# Autodesk Inventor assembly: Pump-Motor-CW-Rotation:Motor CW
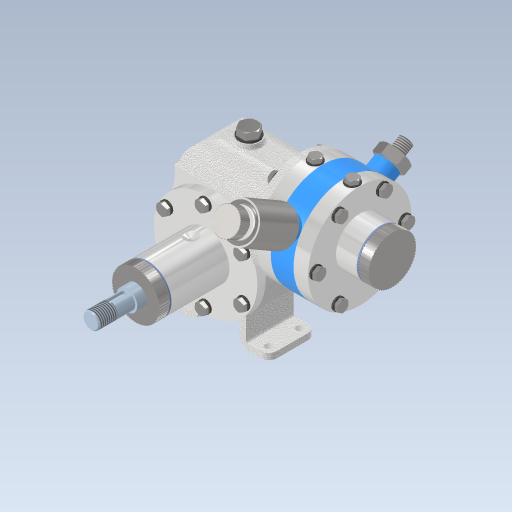
[picture p0: Inventor's stored thumbnail of the model, 512x512]
Saved by Autodesk Inventor 2024.2 (Build 282272000, 272)
## iProperties
Created: 2025-06-16
Document SubType Name: Assembly
Designer: cw
Description: Motor CW
Author: cw
## Documents named in this file (42)
- C:\zWSA2025 TP05 M1\Solution\Motor Final CW.iam
- C:\zWSA2025 TP05 M1\Solution\Motor\Housing.ipt
- C:\zWSA2025 TP05 M1\Solution\Design Accelerator\Worm Gears1.iam
- C:\zWSA2025 TP05 M1\Solution\Motor\Casing 101.ipt
- C:\zWSA2025 TP05 M1\Solution\Motor\Bush.ipt
- C:\zWSA2025 TP05 M1\Solution\Motor\Shaft.ipt
- C:\zWSA2025 TP05 M1\Solution\Motor\Cover 102.ipt
- C:\zWSA2025 TP05 M1\Solution\Motor\Gasket 103.ipt
- C:\zWSA2025 TP05 M1\Solution\Motor\Seal Ring.ipt
- C:\zWSA2025 TP05 M1\Solution\Content Center\en-US\DIN 6885-1 A\DIN 6885 - A 4 x 4 x 25.ipt
- C:\zWSA2025 TP05 M1\Solution\Motor\Washer.ipt
- C:\zWSA2025 TP05 M1\Solution\Motor\Lock Nut.ipt
- C:\zWSA2025\M1\Casing 103 config.ipt
- C:\zWSA2025 TP05 M1\Solution\Content Center\en-US\DIN 3760 A\DIN 3760 - A - 14 x 24 x 7 - NBR.ipt
- C:\zWSA2025 TP05 M1\Solution\Content Center\en-US\DIN 472(1)\DIN 472 - 24 x 1.2.ipt
- C:\zWSA2025 TP05 M1\Solution\Content Center\en-US\DIN 625 SKF(5)\DIN 625 SKF - SKF 6001-2RSH.ipt
- C:\zWSA2025 TP05 M1\Solution\Motor\Spacer.ipt
- C:\zWSA2025 TP05 M1\Solution\Drive Shaft.ipt
- C:\zWSA2025 TP05 M1\Solution\Content Center\en-US\DIN 6885-1 A\DIN 6885 - A 4 x 4 x 28.ipt
- C:\zWSA2025 TP05 M1\Solution\Motor\M Case.ipt
- C:\zWSA2025 TP05 M1\Solution\Content Center\en-US\DIN 6885-1 A\DIN 6885 - A 5 x 5 x 18.ipt
- C:\zWSA2025 TP05 M1\Solution\Motor\Rotor.ipt
- C:\zWSA2025 TP05 M1\Solution\Motor\Vane.ipt
- C:\zWSA2025 TP05 M1\Solution\Content Center\en-US\ISO 8734(2)\ISO 8734 - 5 x 30 - AISO (2).ipt
- C:\zWSA2025\M1\Casing 102 config.ipt
- C:\zWSA2025 TP05 M1\Solution\Motor\Cover 101.ipt
- C:\zWSA2025 TP05 M1\Solution\Motor\Port.ipt
- C:\zWSA2025 TP05 M1\Solution\Motor\S Barrel.ipt
- C:\zWSA2025 TP05 M1\Solution\Motor\Cap 101.ipt
- C:\zWSA2025 TP05 M1\Solution\Content Center\en-US\ISO 4035(2)\ISO 4035 - M12 - ISO.ipt
- C:\zWSA2025 TP05 M1\Solution\Motor\Cap 102.ipt
- C:\zWSA2025 TP05 M1\Solution\Motor\Cover 103.ipt
- C:\zWSA2025 TP05 M1\Solution\Content Center\en-US\ISO 4017(1)\ISO 4017 - M6 x 16 - ISO.ipt
- C:\zWSA2025 TP05 M1\Solution\Content Center\en-US\ISO 7091\ISO 7091 - ST 6 - 100 HV.ipt
- C:\zWSA2025 TP05 M1\Solution\Content Center\en-US\ISO 4017(1)\ISO 4017 - M6 x 30 - ISO.ipt
- C:\zWSA2025 TP05 M1\Solution\Content Center\en-US\ISO 4017(1)\ISO 4017 - M6 x 25 - ISO.ipt
- C:\zWSA2025 TP05 M1\Solution\Motor\Plug 101.ipt
- C:\zWSA2025 TP05 M1\Solution\Motor\Gasket 101.ipt
- C:\zWSA2025 TP05 M1\Solution\Motor\Plug 102.ipt
- C:\zWSA2025 TP05 M1\Solution\Motor\Gasket 102.ipt
- C:\zWSA2025 TP05 M1\Solution\Casing 103 config\Casing 103-cw.ipt
- C:\zWSA2025 TP05 M1\Solution\Casing 102 config\Casing 102-cw.ipt
## Components (88 placed, 39 different names)
1. Housing:1 — Mate:3, Mate:4, Mate:21, Angle:1(RotateDriveDrive), Mate:30, Mate:31, Mate:32, Mate:33, Mate:34, Flush:7(4cw), Mate:61(4ccw), Mate:114, Mate:115, Angle:103, Angle:104, Mate:134, Mate:135, Angle:108, Mate:138, Mate:139, Angle:109, Angle:110(RotateShaft)
2. Worm Gears:1 [sub-assembly] — Flush:2, Mate:26, Mate:30, Mate:31, Mate:45, Flush:5, Mate:53
3. Casing 101:1 — Mate:3, Mate:4, Mate:5, Mate:6, Mate:7, Mate:8, Mate:9, Mate:10, Mate:11, Mate:18, Mate:19, Mate:20, Mate:21, Mate:110, Mate:111, Angle:102
4. Bush:1 — Mate:5, Mate:6, Mate:7
5. Bush:2 — Mate:8, Mate:9, Mate:10, Mate:12
6. Shaft:1 — Mate:11, Mate:12, Mate:22, Mate:23, Mate:24, Flush:2, Mate:25, Mate:27, Mate:28, Angle:110(RotateShaft)
7. Cover 102:1 — Mate:13, Mate:14, Mate:15, Mate:16, Flush:1, Mate:17, Mate:18, Mate:20
8. Gasket 103:1 — Mate:13, Mate:14, Mate:15, Mate:19
9. Seal Ring:1 — Mate:16, Flush:1, Mate:17
10. DIN 6885-1 A A 4 x 4 x 25:1 — Mate:22, Mate:23, Mate:24
11. Washer:1 — Mate:25, Mate:26, Mate:27, Mate:29, Flush:3
12. Lock Nut:1 — Mate:28, Mate:29, Flush:3
13. Casing 103-cw:1 — Mate:32, Mate:33, Mate:34, Mate:38, Mate:39, Mate:41, Flush:4, Mate:40, Mate:43, Mate:44, Mate:58(4cw), Mate:60(4ccw), Mate:79, Mate:80, Mate:118, Mate:119, Mate:126, Mate:127, Angle:106
14. DIN 3760 A A - 14 x 24 x 7 - NBR:1 — Mate:35, Mate:36, Mate:37, Mate:38, Mate:39, Mate:40
15. DIN 3760 A A - 14 x 24 x 7 - NBR:2 — Mate:35, Mate:36, Mate:37, Mate:42
16. DIN 472 24 x 1.2:1 — Mate:41, Mate:42, Flush:4
17. DIN 625 SKF- with two RS1 seals SKF 6001-2RSH:1 — Mate:43, Mate:44, Mate:47, Mate:48, Flush:6
18. Spacer:1 — Mate:46, Mate:47
19. Drive Shaft:1 — Mate:45, Mate:46, Mate:48, Flush:5, Flush:6, Mate:49, Mate:50, Mate:51, Mate:52, Mate:54, Mate:55, Angle:1(RotateDriveDrive), Mate:59(4cw), Flush:8(4ccw), Mate:62, Mate:63, Mate:64, Mate:65(4cw), Flush:9(4cw), Flush:10(4cw), Mate:66(4ccw), Mate:67(4ccw), Mate:68(4ccw), Mate:78, Mate:81, Mate:82, Mate:84, Mate:85, Mate:87
20. DIN 6885-1 A A 4 x 4 x 28:1 — Mate:49, Mate:50, Mate:51
21. Washer:2 — Mate:52, Mate:53, Mate:54, Mate:56, Mate:57
22. Lock Nut:2 — Mate:55, Mate:56, Mate:57
23. M Case:1 — Mate:58(4cw), Mate:59(4cw), Flush:7(4cw), Mate:60(4ccw), Flush:8(4ccw), Mate:61(4ccw), Tangent:1(4cw), Tangent:2 (4ccw), Tangent:3(4cw), Tangent:4(4ccw), Tangent:5(4cw), Tangent:6(4ccw), Tangent:7(4cw), Tangent:8(4ccw), Mate:74, Flush:83, Mate:75, Flush:84, Mate:94, Mate:95, Angle:97, Mate:96, Mate:97, Angle:98, Mate:99
24. DIN 6885-1 A A 5 x 5 x 18:1 — Mate:62, Mate:63, Mate:64
25. Rotor:1 — Mate:65(4cw), Flush:9(4cw), Flush:10(4cw), Mate:66(4ccw), Mate:67(4ccw), Mate:68(4ccw), Flush:70(4cw), Mate:70(4cw), Flush:72(4ccw), Mate:71(4ccw), Flush:73(4cw), Mate:72(4cw), Flush:74(4ccw), Flush:75(4ccw), Flush:76(4cw), Flush:77(4cw), Flush:78(4ccw), Flush:79(4ccw), Flush:80(4cw), Flush:81(4cw), Flush:82(4ccw), Mate:73(4ccw)
26. Vane:1 — Flush:70(4cw), Mate:70(4cw), Tangent:1(4cw), Flush:72(4ccw), Mate:71(4ccw), Tangent:2 (4ccw)
27. Vane:2 — Flush:73(4cw), Mate:72(4cw), Tangent:3(4cw), Flush:74(4ccw), Flush:75(4ccw), Tangent:4(4ccw)
28. Vane:3 — Flush:76(4cw), Flush:77(4cw), Tangent:5(4cw), Flush:78(4ccw), Flush:79(4ccw), Tangent:6(4ccw)
29. Vane:4 — Flush:80(4cw), Flush:81(4cw), Tangent:7(4cw), Flush:82(4ccw), Mate:73(4ccw), Tangent:8(4ccw)
30. ISO 8734 5 x 30 - A:1 — Mate:74, Flush:83
31. ISO 8734 5 x 30 - A:2 — Mate:75, Flush:84
32. Casing 102-cw:1 — Mate:76, Mate:77, Mate:78, Mate:79, Mate:80, Mate:91, Mate:92, Mate:93, Mate:122, Mate:123, Angle:105, Mate:130, Mate:131, Angle:107
33. DIN 625 SKF- with two RS1 seals SKF 6001-2RSH:2 — Mate:76, Mate:77, Mate:81, Mate:83
34. Washer:3 — Mate:82, Mate:83, Mate:84, Mate:86
35. Lock Nut:3 — Mate:85, Mate:86, Mate:87
36. Gasket 103:2 — Mate:88, Mate:89, Mate:90, Mate:92
37. Cover 101:1 — Mate:88, Mate:89, Mate:90, Mate:91, Mate:93
38. Port:1 — Mate:94, Mate:95, Angle:97
39. S Barrel:1 — Mate:96, Mate:97, Angle:98, Mate:98, Mate:100, Angle:99, Mate:102, Mate:103, Angle:100, Mate:104, Mate:106, Angle:101
40. Cap 101:1 — Mate:98, Mate:99, Mate:101
41. ISO 4035 M12:1 — Mate:100, Mate:101, Angle:99
42. ISO 4035 M12:2 — Mate:102, Mate:103, Angle:100, Mate:105
43. Cap 102:1 — Mate:104, Mate:105, Mate:107
44. Cover 103:1 — Mate:106, Mate:107, Angle:101
45. Plug 101:1 — Mate:124, Mate:125, Mate:126, Angle:106
46. Plug 101:2 — Mate:128, Mate:129, Mate:130, Angle:107
47. Gasket 101:1 — Mate:124, Mate:125, Mate:127
48. Gasket 101:2 — Mate:128, Mate:129, Mate:131
49. Plug 102:1 — Mate:132, Mate:133, Mate:134, Angle:108
50. Plug 102:2 — Mate:136, Mate:137, Mate:138, Angle:109
51. Gasket 102:1 — Mate:132, Mate:133, Mate:135
52. Gasket 102:2 — Mate:136, Mate:137, Mate:139
53. ISO 4017 M6 x 16:1 — Mate:108, Mate:109, Mate:110, Angle:102
54. ISO 7091 ST 6 - 100 HV:1 — Mate:108, Mate:109, Mate:111
55. ISO 4017 M6 x 16:2
56. ISO 7091 ST 6 - 100 HV:2
57. ISO 4017 M6 x 16:3
58. ISO 7091 ST 6 - 100 HV:3
59. ISO 4017 M6 x 16:4
60. ISO 7091 ST 6 - 100 HV:4
61. ISO 4017 M6 x 16:5
62. ISO 7091 ST 6 - 100 HV:5
63. ISO 4017 M6 x 16:6
64. ISO 7091 ST 6 - 100 HV:6
65. ISO 4017 M6 x 30:1 — Mate:112, Mate:113, Mate:114, Angle:103
66. ISO 7091 ST 6 - 100 HV:7 — Mate:112, Mate:113, Mate:115
67. ISO 4017 M6 x 30:2
68. ISO 7091 ST 6 - 100 HV:8
69. ISO 4017 M6 x 30:3
70. ISO 7091 ST 6 - 100 HV:9
71. ISO 4017 M6 x 30:4
72. ISO 7091 ST 6 - 100 HV:10
73. ISO 4017 M6 x 25:1 — Mate:116, Mate:117, Mate:118, Angle:104
74. ISO 7091 ST 6 - 100 HV:11 — Mate:116, Mate:117, Mate:119
75. ISO 4017 M6 x 25:2
76. ISO 7091 ST 6 - 100 HV:12
77. ISO 4017 M6 x 25:3 — Mate:120, Mate:121, Mate:122, Angle:105
78. ISO 7091 ST 6 - 100 HV:13 — Mate:120, Mate:121, Mate:123
79. ISO 4017 M6 x 25:4
80. ISO 7091 ST 6 - 100 HV:14
81. ISO 4017 M6 x 25:5
82. ISO 7091 ST 6 - 100 HV:15
83. ISO 4017 M6 x 25:6
84. ISO 7091 ST 6 - 100 HV:16
85. ISO 4017 M6 x 25:7
86. ISO 7091 ST 6 - 100 HV:17
87. ISO 4017 M6 x 25:8
88. ISO 7091 ST 6 - 100 HV:18
## Component patterns: (6 elements, first: ISO 4017 M6 x 16:1 + ISO 7091 ST 6 - 100 HV:1), (4 elements, first: ISO 4017 M6 x 30:1 + ISO 7091 ST 6 - 100 HV:7), (2 elements, first: ISO 4017 M6 x 25:1 + ISO 7091 ST 6 - 100 HV:11), (6 elements, first: ISO 4017 M6 x 25:3 + ISO 7091 ST 6 - 100 HV:13)
## Relationships (183: Mate 136, Flush 24, Angle 15, Tangent 8)
- Mate:3: Housing:1 ↔ Casing 101:1
- Mate:4: Housing:1 ↔ Casing 101:1
- Mate:5: Casing 101:1 ↔ Bush:1
- Mate:6: Casing 101:1 ↔ Bush:1
- Mate:7: Casing 101:1 ↔ Bush:1
- Mate:8: Casing 101:1 ↔ Bush:2
- Mate:9: Casing 101:1 ↔ Bush:2
- Mate:10: Casing 101:1 ↔ Bush:2
- Mate:11: Casing 101:1 ↔ Shaft:1
- Mate:12: Bush:2 ↔ Shaft:1
- Mate:13: Cover 102:1 ↔ Gasket 103:1
- Mate:14: Cover 102:1 ↔ Gasket 103:1
- Mate:15: Cover 102:1 ↔ Gasket 103:1
- Mate:16: Cover 102:1 ↔ Seal Ring:1
- Flush:1 (-3.6 mm): Cover 102:1 ↔ Seal Ring:1
- Mate:17: Cover 102:1 ↔ Seal Ring:1
- Mate:18: Casing 101:1 ↔ Cover 102:1
- Mate:19: Casing 101:1 ↔ Gasket 103:1
- Mate:20: Casing 101:1 ↔ Cover 102:1
- Mate:21: Housing:1 ↔ Casing 101:1
- Mate:22: Shaft:1 ↔ DIN 6885-1 A A 4 x 4 x 25:1
- Mate:23: Shaft:1 ↔ DIN 6885-1 A A 4 x 4 x 25:1
- Mate:24: Shaft:1 ↔ DIN 6885-1 A A 4 x 4 x 25:1
- Flush:2: Worm Gears:1 ↔ Shaft:1
- Flush:6: DIN 625 SKF- with two RS1 seals SKF 6001-2RSH:1 ↔ Drive Shaft:1
- Mate:49: Drive Shaft:1 ↔ DIN 6885-1 A A 4 x 4 x 28:1
- Mate:50: Drive Shaft:1 ↔ DIN 6885-1 A A 4 x 4 x 28:1
- Mate:51: Drive Shaft:1 ↔ DIN 6885-1 A A 4 x 4 x 28:1
- Mate:52: Drive Shaft:1 ↔ Washer:2
- Mate:54: Drive Shaft:1 ↔ Washer:2
- Mate:55: Drive Shaft:1 ↔ Lock Nut:2
- Angle:1(RotateDriveDrive) (0 deg): Housing:1 ↔ Drive Shaft:1
- Mate:25: Shaft:1 ↔ Washer:1
- Mate:26: Worm Gears:1 ↔ Washer:1
- Mate:27: Shaft:1 ↔ Washer:1
- Mate:28: Shaft:1 ↔ Lock Nut:1
- Mate:29: Washer:1 ↔ Lock Nut:1
- Flush:3: Washer:1 ↔ Lock Nut:1
- Mate:30: Housing:1 ↔ Worm Gears:1
- Mate:31: Housing:1 ↔ Worm Gears:1
- Mate:32: Housing:1 ↔ Casing 103-cw:1
- Mate:33: Housing:1 ↔ Casing 103-cw:1
- Mate:34: Housing:1 ↔ Casing 103-cw:1
- Mate:35: DIN 3760 A A - 14 x 24 x 7 - NBR:1 ↔ DIN 3760 A A - 14 x 24 x 7 - NBR:2
- Mate:36: DIN 3760 A A - 14 x 24 x 7 - NBR:1 ↔ DIN 3760 A A - 14 x 24 x 7 - NBR:2
- Mate:37: DIN 3760 A A - 14 x 24 x 7 - NBR:1 ↔ DIN 3760 A A - 14 x 24 x 7 - NBR:2
- Mate:38: Casing 103-cw:1 ↔ DIN 3760 A A - 14 x 24 x 7 - NBR:1
- Mate:39: Casing 103-cw:1 ↔ DIN 3760 A A - 14 x 24 x 7 - NBR:1
- Mate:40: Casing 103-cw:1 ↔ DIN 3760 A A - 14 x 24 x 7 - NBR:1
- Mate:41: Casing 103-cw:1 ↔ DIN 472 24 x 1.2:1
- Mate:42: DIN 3760 A A - 14 x 24 x 7 - NBR:2 ↔ DIN 472 24 x 1.2:1
- Flush:4: Casing 103-cw:1 ↔ DIN 472 24 x 1.2:1
- Mate:43: Casing 103-cw:1 ↔ DIN 625 SKF- with two RS1 seals SKF 6001-2RSH:1
- Mate:44: Casing 103-cw:1 ↔ DIN 625 SKF- with two RS1 seals SKF 6001-2RSH:1
- Mate:45: Worm Gears:1 ↔ Drive Shaft:1
- Mate:46: Spacer:1 ↔ Drive Shaft:1
- Mate:47: DIN 625 SKF- with two RS1 seals SKF 6001-2RSH:1 ↔ Spacer:1
- Mate:48: DIN 625 SKF- with two RS1 seals SKF 6001-2RSH:1 ↔ Drive Shaft:1
- Flush:5: Worm Gears:1 ↔ Drive Shaft:1
- Mate:53: Worm Gears:1 ↔ Washer:2
- Mate:56: Washer:2 ↔ Lock Nut:2
- Mate:57: Washer:2 ↔ Lock Nut:2
- Mate:58(4cw): Casing 103-cw:1 ↔ M Case:1
- Mate:59(4cw): Drive Shaft:1 ↔ M Case:1
- Flush:7(4cw): Housing:1 ↔ M Case:1
- Mate:60(4ccw): Casing 103-cw:1 ↔ M Case:1
- Flush:8(4ccw): Drive Shaft:1 ↔ M Case:1
- Mate:61(4ccw): Housing:1 ↔ M Case:1
- Mate:62: Drive Shaft:1 ↔ DIN 6885-1 A A 5 x 5 x 18:1
- Mate:63: Drive Shaft:1 ↔ DIN 6885-1 A A 5 x 5 x 18:1
- Mate:64: Drive Shaft:1 ↔ DIN 6885-1 A A 5 x 5 x 18:1
- Mate:65(4cw): Drive Shaft:1 ↔ Rotor:1
- Flush:9(4cw): Drive Shaft:1 ↔ Rotor:1
- Flush:10(4cw): Drive Shaft:1 ↔ Rotor:1
- Mate:66(4ccw): Drive Shaft:1 ↔ Rotor:1
- Mate:67(4ccw): Drive Shaft:1 ↔ Rotor:1
- Mate:68(4ccw): Drive Shaft:1 ↔ Rotor:1
- Flush:70(4cw): Rotor:1 ↔ Vane:1
- Mate:70(4cw): Rotor:1 ↔ Vane:1
- Tangent:1(4cw): M Case:1 ↔ Vane:1
- Flush:72(4ccw): Rotor:1 ↔ Vane:1
- Mate:71(4ccw): Rotor:1 ↔ Vane:1
- Tangent:2 (4ccw): M Case:1 ↔ Vane:1
- Flush:73(4cw): Rotor:1 ↔ Vane:2
- Mate:72(4cw): Rotor:1 ↔ Vane:2
- Tangent:3(4cw): M Case:1 ↔ Vane:2
- Flush:74(4ccw): Rotor:1 ↔ Vane:2
- Flush:75(4ccw): Rotor:1 ↔ Vane:2
- Tangent:4(4ccw): M Case:1 ↔ Vane:2
- Flush:76(4cw): Rotor:1 ↔ Vane:3
- Flush:77(4cw): Rotor:1 ↔ Vane:3
- Tangent:5(4cw): M Case:1 ↔ Vane:3
- Flush:78(4ccw): Rotor:1 ↔ Vane:3
- Flush:79(4ccw): Rotor:1 ↔ Vane:3
- Tangent:6(4ccw): M Case:1 ↔ Vane:3
- Flush:80(4cw): Rotor:1 ↔ Vane:4
- Flush:81(4cw): Rotor:1 ↔ Vane:4
- Tangent:7(4cw): M Case:1 ↔ Vane:4
- Flush:82(4ccw): Rotor:1 ↔ Vane:4
- Mate:73(4ccw): Rotor:1 ↔ Vane:4
- Tangent:8(4ccw): M Case:1 ↔ Vane:4
- Mate:74: M Case:1 ↔ ISO 8734 5 x 30 - A:1
- Flush:83 (-4 mm): M Case:1 ↔ ISO 8734 5 x 30 - A:1
- Mate:75: M Case:1 ↔ ISO 8734 5 x 30 - A:2
- Flush:84 (-4 mm): M Case:1 ↔ ISO 8734 5 x 30 - A:2
- Mate:76: Casing 102-cw:1 ↔ DIN 625 SKF- with two RS1 seals SKF 6001-2RSH:2
- Mate:77: Casing 102-cw:1 ↔ DIN 625 SKF- with two RS1 seals SKF 6001-2RSH:2
- Mate:78: Drive Shaft:1 ↔ Casing 102-cw:1
- Mate:79 (22 mm): Casing 103-cw:1 ↔ Casing 102-cw:1
- Mate:80: Casing 103-cw:1 ↔ Casing 102-cw:1
- Mate:81: Drive Shaft:1 ↔ DIN 625 SKF- with two RS1 seals SKF 6001-2RSH:2
- Mate:82: Drive Shaft:1 ↔ Washer:3
- Mate:83: DIN 625 SKF- with two RS1 seals SKF 6001-2RSH:2 ↔ Washer:3
- Mate:84: Drive Shaft:1 ↔ Washer:3
- Mate:85: Drive Shaft:1 ↔ Lock Nut:3
- Mate:86: Washer:3 ↔ Lock Nut:3
- Mate:87: Drive Shaft:1 ↔ Lock Nut:3
- Mate:88: Gasket 103:2 ↔ Cover 101:1
- Mate:89: Gasket 103:2 ↔ Cover 101:1
- Mate:90: Gasket 103:2 ↔ Cover 101:1
- Mate:91: Casing 102-cw:1 ↔ Cover 101:1
- Mate:92: Casing 102-cw:1 ↔ Gasket 103:2
- Mate:93: Casing 102-cw:1 ↔ Cover 101:1
- Mate:94: M Case:1 ↔ Port:1
- Mate:95: M Case:1 ↔ Port:1
- Angle:97 (0 deg): M Case:1 ↔ Port:1
- Mate:96: M Case:1 ↔ S Barrel:1
- Mate:97 (-12 mm): M Case:1 ↔ S Barrel:1
- Angle:98 (0 deg): M Case:1 ↔ S Barrel:1
- Mate:98: S Barrel:1 ↔ Cap 101:1
- Mate:99: M Case:1 ↔ Cap 101:1
- Mate:100: S Barrel:1 ↔ ISO 4035 M12:1
- Mate:101: Cap 101:1 ↔ ISO 4035 M12:1
- Angle:99 (0 deg): S Barrel:1 ↔ ISO 4035 M12:1
- Mate:102: S Barrel:1 ↔ ISO 4035 M12:2
- Mate:103 (-14.5 mm): S Barrel:1 ↔ ISO 4035 M12:2
- Angle:100 (0 deg): S Barrel:1 ↔ ISO 4035 M12:2
- Mate:104: S Barrel:1 ↔ Cap 102:1
- Mate:105: ISO 4035 M12:2 ↔ Cap 102:1
- Mate:106: S Barrel:1 ↔ Cover 103:1
- Mate:107: Cap 102:1 ↔ Cover 103:1
- Angle:101 (0 deg): S Barrel:1 ↔ Cover 103:1
- Mate:108: ISO 4017 M6 x 16:1 ↔ ISO 7091 ST 6 - 100 HV:1
- Mate:109: ISO 4017 M6 x 16:1 ↔ ISO 7091 ST 6 - 100 HV:1
- Mate:110: Casing 101:1 ↔ ISO 4017 M6 x 16:1
- Mate:111: Casing 101:1 ↔ ISO 7091 ST 6 - 100 HV:1
- Angle:102 (0 deg): Casing 101:1 ↔ ISO 4017 M6 x 16:1
- Mate:112: ISO 4017 M6 x 30:1 ↔ ISO 7091 ST 6 - 100 HV:7
- Mate:113: ISO 4017 M6 x 30:1 ↔ ISO 7091 ST 6 - 100 HV:7
- Mate:114: Housing:1 ↔ ISO 4017 M6 x 30:1
- Mate:115: Housing:1 ↔ ISO 7091 ST 6 - 100 HV:7
- Angle:103 (0 deg): Housing:1 ↔ ISO 4017 M6 x 30:1
- Mate:116: ISO 4017 M6 x 25:1 ↔ ISO 7091 ST 6 - 100 HV:11
- Mate:117: ISO 4017 M6 x 25:1 ↔ ISO 7091 ST 6 - 100 HV:11
- Mate:118: Casing 103-cw:1 ↔ ISO 4017 M6 x 25:1
- Mate:119: Casing 103-cw:1 ↔ ISO 7091 ST 6 - 100 HV:11
- Angle:104 (0 deg): Housing:1 ↔ ISO 4017 M6 x 25:1
- Mate:120: ISO 4017 M6 x 25:3 ↔ ISO 7091 ST 6 - 100 HV:13
- Mate:121: ISO 4017 M6 x 25:3 ↔ ISO 7091 ST 6 - 100 HV:13
- Mate:122: Casing 102-cw:1 ↔ ISO 4017 M6 x 25:3
- Mate:123: Casing 102-cw:1 ↔ ISO 7091 ST 6 - 100 HV:13
- Angle:105 (0 deg): Casing 102-cw:1 ↔ ISO 4017 M6 x 25:3
- Mate:124: Plug 101:1 ↔ Gasket 101:1
- Mate:125: Plug 101:1 ↔ Gasket 101:1
- Mate:126: Casing 103-cw:1 ↔ Plug 101:1
- Mate:127: Casing 103-cw:1 ↔ Gasket 101:1
- Angle:106 (0 deg): Casing 103-cw:1 ↔ Plug 101:1
- Mate:128: Plug 101:2 ↔ Gasket 101:2
- Mate:129: Plug 101:2 ↔ Gasket 101:2
- Mate:130: Casing 102-cw:1 ↔ Plug 101:2
- Mate:131: Casing 102-cw:1 ↔ Gasket 101:2
- Angle:107 (0 deg): Casing 102-cw:1 ↔ Plug 101:2
- Mate:132: Plug 102:1 ↔ Gasket 102:1
- Mate:133: Plug 102:1 ↔ Gasket 102:1
- Mate:134: Housing:1 ↔ Plug 102:1
- Mate:135: Housing:1 ↔ Gasket 102:1
- Angle:108 (0 deg): Housing:1 ↔ Plug 102:1
- Mate:136: Plug 102:2 ↔ Gasket 102:2
- Mate:137: Plug 102:2 ↔ Gasket 102:2
- Mate:138: Housing:1 ↔ Plug 102:2
- Mate:139: Housing:1 ↔ Gasket 102:2
- Angle:109 (0 deg): Housing:1 ↔ Plug 102:2
- Angle:110(RotateShaft) (0 deg): Housing:1 ↔ Shaft:1
